# Autodesk Inventor assembly: Pickup Arm Right
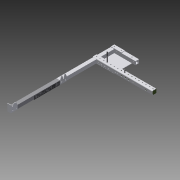
[picture p0: Inventor's stored thumbnail of the model, 180x180]
Saved by Autodesk Inventor 2015 (Build 190159000, 159)
## iProperties
Created: 2015-01-28
Part Number: Pickup Arm Right
Document SubType Name: Assembly
Designer: Admin
Author: Admin
## Documents named in this file (15)
- D:\Robotics\FRC\2015\CAD\Robot\Pickup Arms\Pickup Arm Right.iam
- D:\Robotics\FRC\2015\CAD\Robot\Pickup Arms\rack.ipt
- D:\Robotics\FRC\2015\CAD\Robot\Pickup Arms\1x1 pickup arm support rear.ipt
- D:\Robotics\FRC\2015\CAD\Robot\Pickup Arms\1x1 pickup arm support.ipt
- D:\Robotics\FRC\2015\CAD\Robot\Pickup Arms\pickup arm gusset.ipt
- D:\Robotics\FRC\2015\CAD\Robot\Pickup Arms\pickup arm plate.ipt
- D:\Robotics\FRC\2015\CAD\Robot\Pickup Arms\spacer.ipt
- D:\Robotics\FRC\2015\CAD\Robot\Pickup Arms\mechanical stop bolt.ipt
- D:\Robotics\FRC\2015\CAD\Robot\Pickup Arms\pickup arm 1x1 long.ipt
- D:\Robotics\FRC\2015\CAD\Robot\Pickup Arms\pickup arm tab.ipt
- D:\Robotics\FRC\2015\CAD\Robot\Pickup Arms\C-Channel.ipt
- D:\Robotics\FRC\2015\CAD\Robot\Pickup Arms\rubber grip.ipt
- D:\Robotics\FRC\2015\CAD\Robot\Pickup Arms\beam breaker bolt.ipt
- D:\Robotics\FRC\2015\CAD\Robot\Pickup Arms\front tab 2x2.ipt
- D:\Robotics\FRC\2015\CAD\Robot\Pickup Arms\1x1 angle arm extender.ipt
## Components (14 placed, 14 different names)
1. pickup arm 1x1 long:1 — Mate:19, Flush:2, Mate:20, Mate:21, Flush:3, Flush:4, Flush:5, Mate:22, Flush:6, Mate:23, Mate:26, Flush:10, Flush:12, Mate:32, Mate:37, Mate:38, Mate:39, Mate:42, Mate:46, Mate:47
2. pickup arm plate:1 — Mate:11, Mate:17, Mate:18, Mate:19, Flush:2, Flush:4
3. 1x1 pickup arm support:1 — Mate:11, Flush:3, Mate:22
4. 1x1 pickup arm support rear:1 — Mate:16, Mate:30, Mate:31
5. rack:1 — Mate:16, Mate:28, Mate:29, Flush:13
6. C-Channel:1 — Mate:28, Mate:29, Mate:30, Mate:31, Flush:12, Mate:32, Mate:33, Mate:40, Mate:41, Flush:13
7. pickup arm gusset:1 — Flush:5, Flush:6, Mate:23
8. spacer:1 — Mate:20, Mate:21, Mate:33
9. mechanical stop bolt:1 — Mate:17, Mate:18
10. beam breaker bolt:1 — Mate:40, Mate:41
11. pickup arm tab:2 — Mate:26, Flush:10, Mate:42, Mate:48
12. front tab 2x2:1 — Mate:49, Mate:50, Flush:14
13. rubber grip:1 — Mate:37, Mate:38, Mate:39
14. 1x1 angle arm extender:1 — Mate:46, Mate:47, Mate:48, Mate:49, Mate:50, Flush:14
## Relationships (36: Mate 27, Flush 9)
- Mate:11: pickup arm plate:1 ↔ 1x1 pickup arm support:1
- Mate:16: 1x1 pickup arm support rear:1 ↔ rack:1
- Mate:17: pickup arm plate:1 ↔ mechanical stop bolt:1
- Mate:18: pickup arm plate:1 ↔ mechanical stop bolt:1
- Mate:19: pickup arm 1x1 long:1 ↔ pickup arm plate:1
- Flush:2: pickup arm 1x1 long:1 ↔ pickup arm plate:1
- Mate:20: pickup arm 1x1 long:1 ↔ spacer:1
- Mate:21: pickup arm 1x1 long:1 ↔ spacer:1
- Flush:3: pickup arm 1x1 long:1 ↔ 1x1 pickup arm support:1
- Flush:4: pickup arm 1x1 long:1 ↔ pickup arm plate:1
- Flush:5: pickup arm 1x1 long:1 ↔ pickup arm gusset:1
- Mate:22: pickup arm 1x1 long:1 ↔ 1x1 pickup arm support:1
- Flush:6: pickup arm 1x1 long:1 ↔ pickup arm gusset:1
- Mate:23: pickup arm 1x1 long:1 ↔ pickup arm gusset:1
- Mate:26: pickup arm 1x1 long:1 ↔ pickup arm tab:2
- Flush:10: pickup arm 1x1 long:1 ↔ pickup arm tab:2
- Mate:28: rack:1 ↔ C-Channel:1
- Mate:29 (3.175 mm): rack:1 ↔ C-Channel:1
- Mate:30: 1x1 pickup arm support rear:1 ↔ C-Channel:1
- Mate:31 (3.175 mm): 1x1 pickup arm support rear:1 ↔ C-Channel:1
- Flush:12: pickup arm 1x1 long:1 ↔ C-Channel:1
- Mate:32: pickup arm 1x1 long:1 ↔ C-Channel:1
- Mate:33: C-Channel:1 ↔ spacer:1
- Mate:37: pickup arm 1x1 long:1 ↔ rubber grip:1
- Mate:38: pickup arm 1x1 long:1 ↔ rubber grip:1
- Mate:39: pickup arm 1x1 long:1 ↔ rubber grip:1
- Mate:40: C-Channel:1 ↔ beam breaker bolt:1
- Mate:41: C-Channel:1 ↔ beam breaker bolt:1
- Mate:42: pickup arm 1x1 long:1 ↔ pickup arm tab:2
- Flush:13: rack:1 ↔ C-Channel:1
- Mate:46: pickup arm 1x1 long:1 ↔ 1x1 angle arm extender:1
- Mate:47: pickup arm 1x1 long:1 ↔ 1x1 angle arm extender:1
- Mate:48: pickup arm tab:2 ↔ 1x1 angle arm extender:1
- Mate:49: front tab 2x2:1 ↔ 1x1 angle arm extender:1
- Mate:50: front tab 2x2:1 ↔ 1x1 angle arm extender:1
- Flush:14: front tab 2x2:1 ↔ 1x1 angle arm extender:1
